# Autodesk Inventor assembly: UpperArm
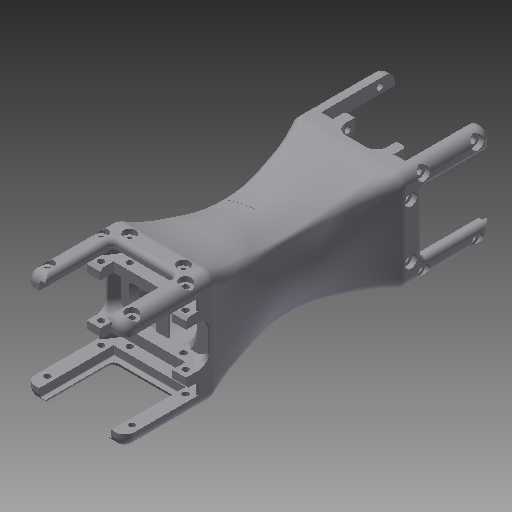
[picture p0: Inventor's stored thumbnail of the model, 512x512]
Saved by Autodesk Inventor 2019 (Build 230136000, 136)
## iProperties
Created: 2019-06-24
Part Number: UpperArm
Document SubType Name: Assembly
Designer: xwermter
Author: xwermter
## Documents named in this file (2)
- Z:\nico\arms\upper_arm.iam
- Z:\nico\arms\upper_arm_half.ipt
## Components (2 placed, 1 different names)
1. upper_arm_half:1 — Mate:1, Mate:2, Angle:1
2. upper_arm_half:2 — Mate:1, Mate:2, Angle:1
## Relationships (3: Mate 2, Angle 1)
- Mate:1: upper_arm_half:1 ↔ upper_arm_half:2
- Mate:2: upper_arm_half:1 ↔ upper_arm_half:2
- Angle:1 (90 deg): upper_arm_half:1 ↔ upper_arm_half:2
